# Autodesk Inventor assembly: TeslaCoil
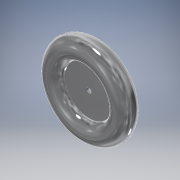
[picture p0: Inventor's stored thumbnail of the model, 180x180]
Saved by Autodesk Inventor 2019 (Build 230136000, 136)
## iProperties
Created: 2020-12-21
Part Number: TeslaCoil
Material: Типовые
Document SubType Name: Assembly
Designer: Dazer
Author: Dazer
## Documents named in this file (2)
- C:\Users\Dazer\Documents\GitHub\Tesla_coil_V1\3dModels\TeslaCoil.iam
- C:\Users\Dazer\Desktop\Toroid.ipt
## Components (2 placed, 1 different names)
1. Toroid:1 — Совмещение:1
2. Toroid:2 — Совмещение:1
## Relationships (1: Mate 1)
- Совмещение:1 [Mate]: Toroid:1 ↔ Toroid:2
